# Autodesk Inventor assembly: UmlenkrolleHalterEinfachAngleB
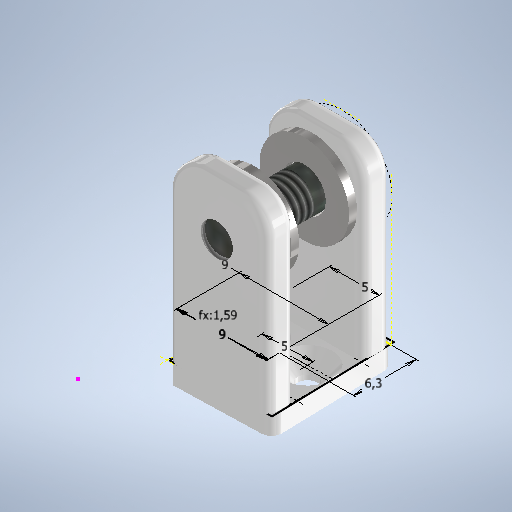
[picture p0: Inventor's stored thumbnail of the model, 512x512]
Saved by Autodesk Inventor 2025 (Build 290162010, 162A)
## iProperties
Created: 2024-11-19
Part Number: UmlenkrolleHalterEinfachAngleB
Document SubType Name: Assembly
Designer: Admin
Mass: 6.79388 g
Surface Area: 35.0539 cm^2
Volume: 2.35136 cm^3
Density: 2.88934 g/cm^3
Author: Admin
## Documents named in this file (5)
- C:\Users\Admin\GIT\HDVKBM\CAD\Krandemonstrator\UmlenkrolleHalterEinfachAngleB.iam
- C:\Users\Admin\GIT\HDVKBM\CAD\Krandemonstrator\Umlenkrolle.iam
- C:\Users\Admin\GIT\HDVKBM\CAD\Krandemonstrator\HalterUmlenkrolleOVR.ipt
- C:\Users\Admin\Documents\Inventor\Content Center Files\R2025\de-DE\DIN EN ISO 7089\DIN EN ISO 7089 -  4.ipt
- C:\Users\Admin\Documents\Inventor\Content Center Files\R2025\de-DE\ISO 10642(2)\ISO 10642  - M4  x  12.ipt
## Components (5 placed, 4 different names)
1. HalterUmlenkrolleOVR:1
2. Umlenkrolle:1 [sub-assembly]
3. DIN EN ISO 7089 4:1
4. DIN EN ISO 7089 4:2
5. DIN EN ISO 10642 M4  x  12:1
## Relationships (4: RevoluteJoint 3, Mate 1)
- [RevoluteJoint]: HalterUmlenkrolleOVR:1 ↔ DIN EN ISO 7089 4:1
- [Mate]: HalterUmlenkrolleOVR:1 ↔ DIN EN ISO 10642 M4  x  12:1
- [RevoluteJoint]: Umlenkrolle:1 ↔ DIN EN ISO 7089 4:1
- [RevoluteJoint]: Umlenkrolle:1 ↔ DIN EN ISO 7089 4:2
